# Autodesk Inventor assembly: Master
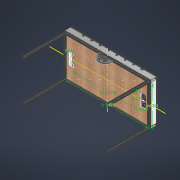
[picture p0: Inventor's stored thumbnail of the model, 180x180]
Saved by Autodesk Inventor 2021 (Build 250183000, 183)
## iProperties
Created: 2021-11-23
Part Number: Master
Document SubType Name: Assembly
Designer: jo_ki
Author: jo_ki
## Documents named in this file (9)
- C:\GIT\SmartSoccerTableCAD\Assemblies\Master.iam
- C:\GIT\SmartSoccerTableCAD\Parts\Beams\leg.ipt
- C:\GIT\SmartSoccerTableCAD\Parts\Beams\tallBeamLong.ipt
- C:\GIT\SmartSoccerTableCAD\Parts\Beams\tallBeamShort.ipt
- C:\GIT\SmartSoccerTableCAD\Parts\Beams\tallBeamLongInlet.ipt
- C:\GIT\SmartSoccerTableCAD\Parts\ballInletWheel.ipt
- C:\GIT\SmartSoccerTableCAD\Parts\Dimensions\Mastersketch.ipt
- C:\GIT\SmartSoccerTableCAD\Parts\Floors\GroundPlate.ipt
- C:\GIT\SmartSoccerTableCAD\Parts\Floors\glassPlate.ipt
## Components (11 placed, 7 different names)
1. leg:1 — Flush:1, Flush:23, Mate:14
2. leg:2 — Flush:14, Flush:15, Mate:8
3. leg:3 — Flush:3, Mate:13, Flush:21, Flush:22
4. leg:4 — Mate:6, Flush:12, Flush:13
5. tallBeamLong:1 — Flush:1, Flush:3, Mate:3, Mate:5, Mate:11, Flush:18, Flush:19, Flush:20, Mate:13, Flush:21, Mate:14
6. tallBeamShort:1 — Mate:5, Flush:15, Flush:16, Flush:20, Flush:22
7. tallBeamShort:2 — Mate:3, Flush:10, Mate:7, Flush:11, Flush:12, Mate:12, Flush:18, Flush:19, Flush:23
8. tallBeamLongInlet:1 — Mate:6, Flush:10, Mate:7, Flush:11, Flush:13, Flush:14, Flush:16, Mate:8, Mate:9, Flush:17, Mate:10, Mate:16
9. ballInletWheel:1 — Mate:9, Flush:17
10. glassPlate:1 — Mate:15, Mate:16, Flush:29
11. GroundPlate:1 — Mate:10, Mate:11, Mate:12, Mate:15, Flush:29
## Relationships (30: Flush 17, Mate 13)
- Flush:1: leg:1 ↔ tallBeamLong:1
- Flush:3: leg:3 ↔ tallBeamLong:1
- Mate:3: tallBeamLong:1 ↔ tallBeamShort:2
- Mate:5: tallBeamLong:1 ↔ tallBeamShort:1
- Mate:6: leg:4 ↔ tallBeamLongInlet:1
- Flush:10: tallBeamShort:2 ↔ tallBeamLongInlet:1
- Mate:7: tallBeamShort:2 ↔ tallBeamLongInlet:1
- Flush:11: tallBeamShort:2 ↔ tallBeamLongInlet:1
- Flush:12: leg:4 ↔ tallBeamShort:2
- Flush:13: leg:4 ↔ tallBeamLongInlet:1
- Flush:14: leg:2 ↔ tallBeamLongInlet:1
- Flush:15: leg:2 ↔ tallBeamShort:1
- Flush:16: tallBeamShort:1 ↔ tallBeamLongInlet:1
- Mate:8: leg:2 ↔ tallBeamLongInlet:1
- Mate:9: tallBeamLongInlet:1 ↔ ballInletWheel:1
- Flush:17 (4.5 mm): tallBeamLongInlet:1 ↔ ballInletWheel:1
- Mate:10: tallBeamLongInlet:1 ↔ GroundPlate:1
- Mate:11 (-11 mm): tallBeamLong:1 ↔ GroundPlate:1
- Mate:12 (-11 mm): tallBeamShort:2 ↔ GroundPlate:1
- Flush:18: tallBeamLong:1 ↔ tallBeamShort:2
- Flush:19: tallBeamLong:1 ↔ tallBeamShort:2
- Flush:20: tallBeamLong:1 ↔ tallBeamShort:1
- Mate:13: leg:3 ↔ tallBeamLong:1
- Flush:21: leg:3 ↔ tallBeamLong:1
- Flush:22: leg:3 ↔ tallBeamShort:1
- Flush:23: leg:1 ↔ tallBeamShort:2
- Mate:14: leg:1 ↔ tallBeamLong:1
- Mate:15: glassPlate:1 ↔ GroundPlate:1
- Mate:16: tallBeamLongInlet:1 ↔ glassPlate:1
- Flush:29: glassPlate:1 ↔ GroundPlate:1
## Named parameters: profile_width = 40 mm, feet_widthCenter = 720 mm, feet_lengthCenter = 1500 mm, feet_length = 746 mm, profile_height = 160 mm, groundPlate_width = 702 mm, groundPlate_length = 1482 mm, handle_distance = 150 mm, handle_amount = 8, handle_offsetTop = 45 mm, handleAxle_diameter = 16 mm, handleHole_diameter = 36 mm, profileTall_innerHeightOffset = 33 mm, profileTallWall_thickness = 3 mm, groundPlate_thickness = 8 mm, ball_size = 33 mm, ball_rollTolerance = 1 mm, glass_thickness = 6 mm, glass_length = 1200 mm, ballInletHole_groundPlateOffsetBottom = 24 mm, ballInletWheel_margin = 10 mm, ballInletWheel_thickness = 31 mm, ballInletWheelBucket_amount = 6, ballInletWheelSlope_angle = 10 deg, goal_width = 224 mm, goal_height = 96 mm, goal_depth = 89 mm, goalCollector_depth = 68 mm, ballRollbackRail_angle = 5 deg, handleAxle_length = 1100 mm, ballInletWheelDriveShaftAxle_diameter = 10 mm, ballInletWheel_diameter = 238.29764 mm, ballInletWheel_offsetTop = 174.68268 mm, ballInletWheel_tolerance = 1 mm
